# Autodesk Inventor assembly: Итоговая сборка
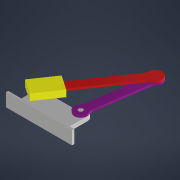
[picture p0: Inventor's stored thumbnail of the model, 180x180]
Saved by Autodesk Inventor 2021.2 (Build 252289000, 289)
## iProperties
Created: 2021-05-30
Part Number: Итоговая сборка
Document SubType Name: Assembly
Designer: Admin
Author: Admin
## Documents named in this file (5)
- D:\Studying\BMSTU Studing\4 term\Applied mechanics\HM2\Модель\Итоговая сборка.iam
- D:\Studying\BMSTU Studing\4 term\Applied mechanics\HM2\Модель\Base.ipt
- D:\Studying\BMSTU Studing\4 term\Applied mechanics\HM2\Модель\Рычаг_1.ipt
- D:\Studying\BMSTU Studing\4 term\Applied mechanics\HM2\Модель\Рычаг_2.ipt
- D:\Studying\BMSTU Studing\4 term\Applied mechanics\HM2\Модель\Каменъ.ipt
## Components (4 placed, 4 different names)
1. Base:1 — С поворотом:1, С поворотом:3
2. Рычаг_1:1 — С поворотом:1, С поворотом:2
3. Рычаг_2:1 — С поворотом:2, Ползун:1
4. Каменъ:1 — С поворотом:3, Ползун:1
## Relationships (4: RevoluteJoint 3, TranslationJoint 1)
- С поворотом:1 [RevoluteJoint]: Base:1 ↔ Рычаг_1:1
- С поворотом:2 [RevoluteJoint]: Рычаг_1:1 ↔ Рычаг_2:1
- С поворотом:3 [RevoluteJoint]: Base:1 ↔ Каменъ:1
- Ползун:1 [TranslationJoint]: Рычаг_2:1 ↔ Каменъ:1
